# Autodesk Inventor assembly: thigh_right
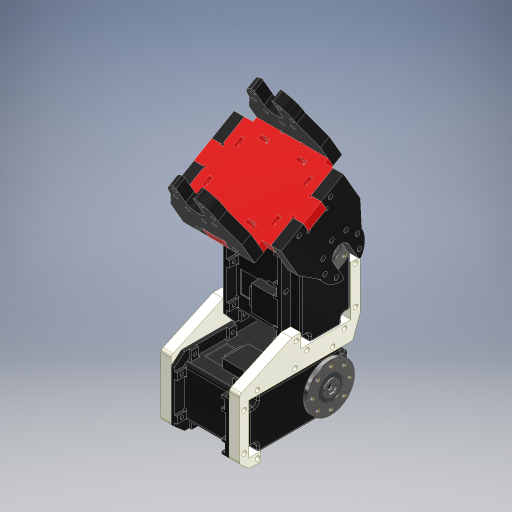
[picture p0: Inventor's stored thumbnail of the model, 512x512]
Saved by Autodesk Inventor 2024 (Build 280153000, 153)
## iProperties
Created: 2024-09-15
Part Number: thigh_right
Document SubType Name: Assembly
Designer: msi
Author: msi
## Documents named in this file (8)
- C:\Users\msi\GITHUB\19th_intern_kgh_fight_robot\부품\Lower_Body\Thigh\thigh_right.iam
- C:\Users\msi\GITHUB\19th_intern_kgh_fight_robot\부품\Lower_Body\Thigh\64_106 fixation.ipt
- C:\Users\msi\GITHUB\19th_intern_kgh_fight_robot\부품\Lower_Body\Thigh\knee fixation.ipt
- C:\Users\msi\GITHUB\19th_intern_kgh_fight_robot\부품\Lower_Body\Thigh\hip joint and thigh connection_106.ipt
- C:\Users\msi\GITHUB\19th_intern_kgh_fight_robot\부품\Lower_Body\Thigh\hip joint nad thigh connection_64.ipt
- C:\Users\msi\GITHUB\19th_intern_kgh_fight_robot\부품\ROBOTIS(Inventor 2024 ver.)\다이나믹셀\MX-106T+idle.ipt.iam
- C:\Users\msi\GITHUB\19th_intern_kgh_fight_robot\부품\ROBOTIS(Inventor 2024 ver.)\혼\64-106Horn.ipt
- MX-106T+idle.ipt
## Components (11 placed, 6 different names)
1. knee fixation:1 — 삽입:23, 삽입:24, 삽입:25, 삽입:26
2. hip joint and thigh connection_106:1 — 삽입:9, 삽입:10, 삽입:18
3. hip joint nad thigh connection_64:1 — 삽입:13, 삽입:14, 각도:1
4. 64_106 fixation:1 — 삽입:9, 삽입:10, 삽입:11, 삽입:12, 삽입:13, 삽입:14, 삽입:15, 삽입:16
5. knee fixation:2 — 삽입:21, 삽입:22, 삽입:27, 삽입:28
6. hip joint and thigh connection_106:2 — 삽입:11, 삽입:12, 삽입:19, 삽입:20
7. hip joint nad thigh connection_64:2 — 삽입:15, 삽입:16
8. MX-106T+idle.ipt:1 [sub-assembly] — 삽입:17, 삽입:18, 삽입:21, 삽입:22, 삽입:23, 삽입:24, 각도:1
9. 64-106Horn:1 — 삽입:17, 삽입:19, 삽입:20
10. MX-106T+idle.ipt:2 [sub-assembly] — 삽입:25, 삽입:26, 삽입:27, 삽입:28, 삽입:29
11. 64-106Horn:2 — 삽입:29
## Relationships (22: Insert 21, Angle 1)
- 삽입:9 [Insert]: hip joint and thigh connection_106:1 ↔ 64_106 fixation:1
- 삽입:10 [Insert]: hip joint and thigh connection_106:1 ↔ 64_106 fixation:1
- 삽입:11 [Insert]: 64_106 fixation:1 ↔ hip joint and thigh connection_106:2
- 삽입:12 [Insert]: 64_106 fixation:1 ↔ hip joint and thigh connection_106:2
- 삽입:13 [Insert]: hip joint nad thigh connection_64:1 ↔ 64_106 fixation:1
- 삽입:14 [Insert]: hip joint nad thigh connection_64:1 ↔ 64_106 fixation:1
- 삽입:15 [Insert]: 64_106 fixation:1 ↔ hip joint nad thigh connection_64:2
- 삽입:16 [Insert]: 64_106 fixation:1 ↔ hip joint nad thigh connection_64:2
- 삽입:17 [Insert]: MX-106T+idle.ipt:1 ↔ 64-106Horn:1
- 삽입:18 [Insert]: hip joint and thigh connection_106:1 ↔ MX-106T+idle.ipt:1
- 삽입:19 [Insert]: hip joint and thigh connection_106:2 ↔ 64-106Horn:1
- 삽입:20 [Insert]: hip joint and thigh connection_106:2 ↔ 64-106Horn:1
- 삽입:21 [Insert]: knee fixation:2 ↔ MX-106T+idle.ipt:1
- 삽입:22 [Insert]: knee fixation:2 ↔ MX-106T+idle.ipt:1
- 삽입:23 [Insert]: knee fixation:1 ↔ MX-106T+idle.ipt:1
- 삽입:24 [Insert]: knee fixation:1 ↔ MX-106T+idle.ipt:1
- 삽입:25 [Insert]: knee fixation:1 ↔ MX-106T+idle.ipt:2
- 삽입:26 [Insert]: knee fixation:1 ↔ MX-106T+idle.ipt:2
- 삽입:27 [Insert]: knee fixation:2 ↔ MX-106T+idle.ipt:2
- 삽입:28 [Insert]: knee fixation:2 ↔ MX-106T+idle.ipt:2
- 삽입:29 [Insert]: MX-106T+idle.ipt:2 ↔ 64-106Horn:2
- 각도:1 [Angle] (-30 deg): hip joint nad thigh connection_64:1 ↔ MX-106T+idle.ipt:1
